# Autodesk Inventor assembly: FUN BLAST
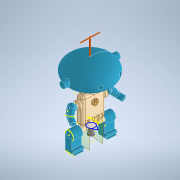
[picture p0: Inventor's stored thumbnail of the model, 180x180]
Saved by Autodesk Inventor 2021 (Build 250183000, 183)
## iProperties
Created: 2021-07-26
Part Number: FUN BLAST
Document SubType Name: Assembly
Designer: user
Author: user
## Documents named in this file (9)
- D:\FINAL ROBO\FUN BLAST.iam
- D:\FINAL ROBO\ROBO BODY PART 1.ipt
- D:\Engineering Exploration\ALL PARTS UNSCALED\toy hand part 2 - Copy.ipt
- D:\Engineering Exploration\ALL PARTS UNSCALED\toy hand part 2.ipt
- D:\FINAL ROBO\HEAD FINAL.ipt
- D:\FINAL ROBO\LEG FINAL 1.ipt
- D:\FINAL ROBO\LEG FINAL 2.ipt
- D:\FINAL ROBO\BASE ROTATING.ipt
- D:\FINAL ROBO\HEAD SHAFT #3434.ipt
## Components (8 placed, 8 different names)
1. ROBO BODY PART 1:1 — Mate:1, Rotational:8, Rotational:9, Rotational:10, Rotational:11, Rotational:12
2. HEAD FINAL:1 — Mate:1, Rotational:13
3. HEAD SHAFT #3434:1 — Rotational:13
4. BASE ROTATING:1 — Rotational:8
5. LEG FINAL 1:1 — Rotational:11
6. LEG FINAL 2:1 — Rotational:12
7. toy hand part 2 - Copy:1 — Rotational:9
8. toy hand part 2:1 — Rotational:10
## Relationships (7: RevoluteJoint 6, Mate 1)
- Mate:1: ROBO BODY PART 1:1 ↔ HEAD FINAL:1
- Rotational:8 [RevoluteJoint]: ROBO BODY PART 1:1 ↔ BASE ROTATING:1
- Rotational:9 [RevoluteJoint]: ROBO BODY PART 1:1 ↔ toy hand part 2 - Copy:1
- Rotational:10 [RevoluteJoint]: ROBO BODY PART 1:1 ↔ toy hand part 2:1
- Rotational:11 [RevoluteJoint]: ROBO BODY PART 1:1 ↔ LEG FINAL 1:1
- Rotational:12 [RevoluteJoint]: ROBO BODY PART 1:1 ↔ LEG FINAL 2:1
- Rotational:13 [RevoluteJoint]: HEAD FINAL:1 ↔ HEAD SHAFT #3434:1
